# Autodesk Inventor assembly: Outer Channel
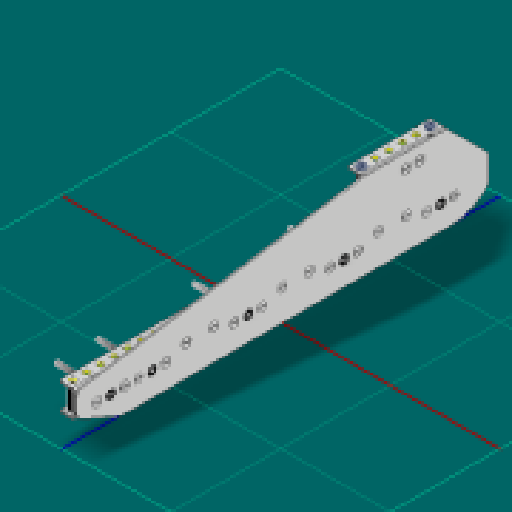
[picture p0: Inventor's stored thumbnail of the model, 512x512]
Saved by Autodesk Inventor 2025 (Build 290162000, 162)
## iProperties
Created: 2024-10-17
Part Number: Outer Channel
Document SubType Name: Assembly
Designer: averey
Author: averey
## Documents named in this file (22)
- C:\Users\avere\VEX\High Stakes\CAD\V2\Chassis\Drivebay Left\Outer Channel.iam
- C:\Users\avere\VEX\High Stakes\CAD\ROBOPROS-CAD-Inventor\Structure\C Channel\Aluminum 1x2x1\Alu C 1x2x1x30.ipt
- C:\Users\avere\VEX\High Stakes\CAD\ROBOPROS-CAD-Inventor\Quick Assemblies\Bearing Flat NScrew Slotted.iam
- C:\Users\avere\VEX\High Stakes\CAD\ROBOPROS-CAD-Inventor\Structure\Hardware\Screw Alloy Steel - Hex\ASScrew Hex Threaded 2.000.ipt
- C:\Users\avere\VEX\High Stakes\CAD\ROBOPROS-CAD-Inventor\Structure\C Channel\Aluminum 1x2x1\Alu C 1x2x1x6.ipt
- C:\Users\avere\VEX\High Stakes\CAD\ROBOPROS-CAD-Inventor\Motion\Spacers\Spacer Nylon .500 OD\NSpacer White .500 OD x .500.ipt
- C:\Users\avere\VEX\High Stakes\CAD\ROBOPROS-CAD-Inventor\Quick Assemblies\Bearing Flat NScrew Slotted Offset.iam
- C:\Users\avere\VEX\High Stakes\CAD\V2\Chassis\Drivebay Left\Custom Parts\Skirt.ipt
- C:\Users\avere\VEX\High Stakes\CAD\ROBOPROS-CAD-Inventor\Motion\Spacers\Spacer Nylon .375 OD\NSpacer .375 OD x .875.ipt
- C:\Users\avere\VEX\High Stakes\CAD\ROBOPROS-CAD-Inventor\Structure\Hardware\Nut Keps.ipt
- C:\Users\avere\VEX\High Stakes\CAD\ROBOPROS-CAD-Inventor\Structure\Standoff\Standoff .875.ipt
- C:\Users\avere\VEX\High Stakes\CAD\ROBOPROS-CAD-Inventor\Structure\Hardware\Screw Steel - Star\SScrew Star Smooth 1.750.ipt
- C:\Users\avere\VEX\High Stakes\CAD\ROBOPROS-CAD-Inventor\Structure\Hardware\Screw Steel - Star\SScrew Star Smooth .290.ipt
- C:\Users\avere\VEX\High Stakes\CAD\ROBOPROS-CAD-Inventor\Motion\Shaft LS\Bearing Flat Low Profile.ipt
- C:\Users\avere\VEX\High Stakes\CAD\ROBOPROS-CAD-Inventor\Structure\Hardware\Screw Shoulder Robosource\SScrew Shoulder Smooth 2.000 x .04.ipt
- C:\Users\avere\VEX\High Stakes\CAD\ROBOPROS-CAD-Inventor\Structure\Hardware\Nut Nylon\Nut Nylon - White.ipt
- C:\Users\avere\VEX\High Stakes\CAD\ROBOPROS-CAD-Inventor\Motion\Spacers\Spacer Nylon .500 OD.ipt
- C:\Users\avere\VEX\High Stakes\CAD\ROBOPROS-CAD-Inventor\Motion\Spacers\Spacer Nylon .375 OD.ipt
- C:\Users\avere\VEX\High Stakes\CAD\ROBOPROS-CAD-Inventor\Structure\Standoff.ipt
- C:\Users\avere\VEX\High Stakes\CAD\ROBOPROS-CAD-Inventor\Structure\Hardware\Screw Steel - Star.ipt
- C:\Users\avere\VEX\High Stakes\CAD\ROBOPROS-CAD-Inventor\Structure\Hardware\Screw Shoulder Robosource.ipt
- C:\Users\avere\VEX\High Stakes\CAD\ROBOPROS-CAD-Inventor\Structure\Hardware\Nut Nylon.ipt
## Components (30 placed, 15 different names)
1. Bearing Flat NScrew Slotted Offset:1 [sub-assembly] — Insert:27, Mate:10
2. Skirt:1 — Insert:12
3. NSpacer .375 OD x .875:1 — Insert:13
4. Nut Keps:1 — Insert:16
5. Nut Keps:2 — Insert:15
6. Standoff .875:1 — Insert:17
7. SScrew Star Smooth 1.750:1 — Insert:18
8. SScrew Star Smooth .290:2 — Insert:19
9. Standoff .875:2 — Insert:22
10. Bearing Flat Low Profile:1 — Insert:23, Mate:9, Insert:25, Insert:26
11. SScrew Shoulder Smooth 2.000 x .04:1 — Insert:24
12. Nut Nylon - White:1 — Insert:25
13. Nut Nylon - White:2 — Insert:26
14. Alu C 1x2x1x30:1 — Mate:1, Insert:3, Mate:4, Insert:4, Mate:5, Insert:5, Mate:6, Insert:6, Insert:7, Insert:9, Insert:10, Insert:15, Insert:16, Insert:18, Insert:22, Insert:23, Mate:9
15. Alu C 1x2x1x6:1 — Insert:13, Insert:17, Insert:19, Insert:24, Insert:27, Mate:10
16. NSpacer White .500 OD x .500:1 — Insert:9
17. NSpacer White .500 OD x .500:2 — Insert:10
18. Bearing Flat NScrew Slotted:3 [sub-assembly] — Insert:4, Mate:5
19. Bearing Flat NScrew Slotted:7 [sub-assembly]
20. Bearing Flat NScrew Slotted:8 [sub-assembly]
21. Bearing Flat NScrew Slotted:1 [sub-assembly] — Insert:3, Mate:4
22. Bearing Flat NScrew Slotted:6 [sub-assembly]
23. ASScrew Hex Threaded 2.000:1 — Insert:6, Insert:12
24. ASScrew Hex Threaded 2.000:2
25. ASScrew Hex Threaded 2.000:3 — Insert:7
26. ASScrew Hex Threaded 2.000:4
27. ASScrew Hex Threaded 2.000:5
28. Bearing Flat NScrew Slotted:9 [sub-assembly] — Insert:5, Mate:6
29. Bearing Flat NScrew Slotted:10 [sub-assembly]
30. Bearing Flat NScrew Slotted:11 [sub-assembly]
## Component patterns: Motor Bearings (3 elements), Front Bearings (2 elements), Front Screw Joints (2 elements), Wheel Screw Joints (3 elements), Wheel Bearings (3 elements)
## Relationships (28: Insert 21, Mate 7)
- Mate:1: Alu C 1x2x1x30:1
- Insert:3: Alu C 1x2x1x30:1 ↔ Bearing Flat NScrew Slotted:1
- Mate:4: Alu C 1x2x1x30:1 ↔ Bearing Flat NScrew Slotted:1
- Insert:4: Alu C 1x2x1x30:1 ↔ Bearing Flat NScrew Slotted:3
- Mate:5: Alu C 1x2x1x30:1 ↔ Bearing Flat NScrew Slotted:3
- Insert:5: Alu C 1x2x1x30:1 ↔ Bearing Flat NScrew Slotted:9
- Mate:6: Alu C 1x2x1x30:1 ↔ Bearing Flat NScrew Slotted:9
- Insert:6 (-1.5875 mm): Alu C 1x2x1x30:1 ↔ ASScrew Hex Threaded 2.000:1
- Insert:7 (-1.5875 mm): Alu C 1x2x1x30:1 ↔ ASScrew Hex Threaded 2.000:3
- [Insert]: Alu C 1x2x1x6:1 ↔ NSpacer White .500 OD x .500:1
- [Mate]: Alu C 1x2x1x6:1 ↔ NSpacer White .500 OD x .500:2
- Insert:9: Alu C 1x2x1x30:1 ↔ NSpacer White .500 OD x .500:1
- Insert:10: Alu C 1x2x1x30:1 ↔ NSpacer White .500 OD x .500:2
- Insert:12: Skirt:1 ↔ ASScrew Hex Threaded 2.000:1
- Insert:13: NSpacer .375 OD x .875:1 ↔ Alu C 1x2x1x6:1
- Insert:15: Nut Keps:2 ↔ Alu C 1x2x1x30:1
- Insert:16: Nut Keps:1 ↔ Alu C 1x2x1x30:1
- Insert:17: Standoff .875:1 ↔ Alu C 1x2x1x6:1
- Insert:18: SScrew Star Smooth 1.750:1 ↔ Alu C 1x2x1x30:1
- Insert:19: SScrew Star Smooth .290:2 ↔ Alu C 1x2x1x6:1
- Insert:22: Standoff .875:2 ↔ Alu C 1x2x1x30:1
- Insert:23: Bearing Flat Low Profile:1 ↔ Alu C 1x2x1x30:1
- Mate:9: Bearing Flat Low Profile:1 ↔ Alu C 1x2x1x30:1
- Insert:24: SScrew Shoulder Smooth 2.000 x .04:1 ↔ Alu C 1x2x1x6:1
- Insert:25 (1.27 mm): Bearing Flat Low Profile:1 ↔ Nut Nylon - White:1
- Insert:26 (1.27 mm): Bearing Flat Low Profile:1 ↔ Nut Nylon - White:2
- Insert:27: Bearing Flat NScrew Slotted Offset:1 ↔ Alu C 1x2x1x6:1
- Mate:10: Bearing Flat NScrew Slotted Offset:1 ↔ Alu C 1x2x1x6:1
## Named parameters: d42_d41 = 0 mm
